# Autodesk Inventor assembly: ORB
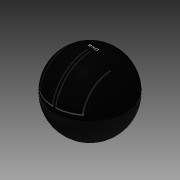
[picture p0: Inventor's stored thumbnail of the model, 180x180]
Saved by Autodesk Inventor 2015 (Build 190159000, 159)
## iProperties
Created: 2014-12-21
Part Number: ORB
Document SubType Name: Assembly
Designer: Sudhar
Author: Sudhar
## Documents named in this file (3)
- C:\Users\Sudhar\Computer Documents\Desktop\ORB\ORB.iam
- C:\Users\Sudhar\Computer Documents\Desktop\ORB\ORB-bottom.ipt
- C:\Users\Sudhar\Computer Documents\Desktop\ORB\ORB-top.ipt
## Components (2 placed, 2 different names)
1. ORB-bottom:1 — Mate:1
2. ORB-top:1 — Mate:1
## Relationships (1: Mate 1)
- Mate:1: ORB-bottom:1 ↔ ORB-top:1
